# Autodesk Inventor assembly: zlozenie_podwozie
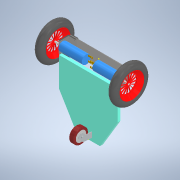
[picture p0: Inventor's stored thumbnail of the model, 180x180]
Saved by Autodesk Inventor 2022 (Build 260153000, 153)
## iProperties
Created: 2023-08-06
Part Number: zlozenie_podwozie
Document SubType Name: Assembly
Designer: Admin
Author: Admin
## Documents named in this file (8)
- C:\Users\Admin\Documents\Inventor\projekcik wakacyjny\zlozenie_podwozie.iam
- C:\Users\Admin\Documents\Inventor\projekcik wakacyjny\blaszka z tylu.ipt
- C:\Users\Admin\Documents\Inventor\projekcik wakacyjny\katownik przedni.ipt
- C:\Users\Admin\Documents\Inventor\projekcik wakacyjny\katownik boczny.ipt
- C:\Users\Admin\Documents\Inventor\projekcik wakacyjny\silniczek.ipt
- C:\Users\Admin\Documents\Inventor\projekcik wakacyjny\podloga_druk.ipt
- C:\Users\Admin\Documents\Inventor\projekcik wakacyjny\kolo_tylne_male.ipt
- C:\Users\Admin\Documents\Inventor\projekcik wakacyjny\nowe_przednie_male.ipt
## Components (11 placed, 7 different names)
1. blaszka z tylu:1 — Mate:1, Mate:2, Mate:3, Rotational:1
2. katownik przedni:1 — Mate:1
3. katownik przedni:2 — Mate:2, Mate:4, Mate:5
4. katownik boczny:2 — Mate:3, Rotational:2
5. katownik boczny:3 — Rotational:1, Rotational:3
6. silniczek:1 — Rotational:2, Insert:1
7. silniczek:2 — Rotational:3, Mate:7
8. podloga_druk:1 — Mate:4, Mate:5, Mate:8
9. kolo_tylne_male:1 — Insert:1
10. kolo_tylne_male:2 — Mate:7
11. nowe_przednie_male:1 — Mate:8
## Relationships (11: Mate 7, RevoluteJoint 3, Insert 1)
- Mate:1: blaszka z tylu:1 ↔ katownik przedni:1
- Mate:2: blaszka z tylu:1 ↔ katownik przedni:2
- Mate:3: blaszka z tylu:1 ↔ katownik boczny:2
- Rotational:1 [RevoluteJoint]: blaszka z tylu:1 ↔ katownik boczny:3
- Rotational:2 [RevoluteJoint] (4 mm): katownik boczny:2 ↔ silniczek:1
- Rotational:3 [RevoluteJoint] (4 mm): katownik boczny:3 ↔ silniczek:2
- Mate:4: katownik przedni:2 ↔ podloga_druk:1
- Mate:5: katownik przedni:2 ↔ podloga_druk:1
- Mate:7: silniczek:2 ↔ kolo_tylne_male:2
- Insert:1: silniczek:1 ↔ kolo_tylne_male:1
- Mate:8: podloga_druk:1 ↔ nowe_przednie_male:1
